# Autodesk Inventor assembly: chassis
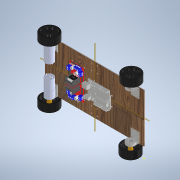
[picture p0: Inventor's stored thumbnail of the model, 180x180]
Saved by Autodesk Inventor 2022 (Build 260153000, 153)
## iProperties
Created: 2023-03-16
Part Number: chassis
Document SubType Name: Assembly
Designer: JOU
Author: JOU
## Documents named in this file (13)
- C:\Users\Johnny Jou\Documents\GitHub\Areo_Rider_Cabin\car\chassis.iam
- C:\Users\Johnny Jou\Documents\GitHub\Areo_Rider_Cabin\car\base.ipt
- C:\Users\Johnny Jou\Documents\GitHub\Areo_Rider_Cabin\car\motor_base.ipt
- C:\Users\Johnny Jou\Documents\GitHub\Areo_Rider_Cabin\motor\25GA370.ipt
- C:\Users\Johnny Jou\Documents\GitHub\Areo_Rider_Cabin\car\Coupling.ipt
- C:\Users\Johnny Jou\Documents\GitHub\Areo_Rider_Cabin\car\wheel.ipt
- C:\Users\Johnny Jou\Documents\GitHub\Areo_Rider_Cabin\car\chassis\機械便覽魔法師\軸承1.iam
- C:\Users\Johnny Jou\Documents\GitHub\Areo_Rider_Cabin\car\axle 4_20.ipt
- C:\Users\Johnny Jou\Documents\GitHub\Areo_Rider_Cabin\car\wheel_base.ipt
- C:\Users\Johnny Jou\Documents\GitHub\Areo_Rider_Cabin\car\wheel_base_cover.ipt
- C:\Users\Johnny Jou\Documents\GitHub\Areo_Rider_Cabin\car\arduino uno.ipt
- C:\Users\Johnny Jou\Documents\GitHub\Areo_Rider_Cabin\car\L298N.ipt
- C:\Users\Johnny Jou\Documents\GitHub\Areo_Rider_Cabin\car\bearing.iam
## Components (25 placed, 11 different names)
1. base:1 — 貼合:1, 貼合:2, 貼合:5, 貼合:6, 貼合:7, 貼合:8, 貼合:78, 貼合:79, 貼合:80, 貼合:81, 貼合:82, 貼合:83, 貼合:84, 貼合:85, 貼合:86, 貼合:87, 貼合:88, 貼合:89, 貼合:90, 貼合:91, 貼合:92
2. motor_base:1 — 貼合:1, 貼合:5, 貼合:6, 貼合:16, 貼合:17, 貼合:18
3. motor_base:2 — 貼合:2, 貼合:7, 貼合:8, 貼合:13, 貼合:14, 貼合:15
4. 25GA370:1 — 貼合:13, 貼合:14, 貼合:15, 貼合:33, 貼合:34
5. 25GA370:3 — 貼合:16, 貼合:17, 貼合:18, 貼合:22, 貼合:23
6. Coupling:1 — 貼合:19, 貼合:20, 貼合:21, 貼合:22, 貼合:23
7. wheel:1 — 貼合:19, 貼合:20, 貼合:21
8. Coupling:4 — 貼合:33, 貼合:34
9. wheel:4
10. Coupling:6 — 貼合:95
11. wheel:6
12. axle 4_20:3 — 貼合:93, 齊平:5
13. wheel_base:3 — 貼合:78, 貼合:82, 貼合:83
14. wheel_base_cover:3 — 貼合:94, 貼合:96
15. Coupling:7 — 貼合:98
16. wheel:7
17. 軸承:4 [sub-assembly]
18. axle 4_20:4 — 貼合:97, 齊平:6
19. wheel_base:4 — 貼合:79, 貼合:80, 貼合:81, 貼合:100, 貼合:102, 貼合:103
20. wheel_base_cover:4 — 貼合:99, 貼合:100, 貼合:101, 貼合:102, 貼合:103
21. arduino uno:1 — 貼合:84, 貼合:85, 貼合:86
22. L298N:1 — 貼合:87, 貼合:91, 貼合:92
23. L298N:2 — 貼合:88, 貼合:89, 貼合:90
24. 軸承:5 [sub-assembly] — 貼合:93, 齊平:5, 貼合:94, 貼合:95, 貼合:96
25. 軸承:6 [sub-assembly] — 貼合:97, 齊平:6, 貼合:98, 貼合:99, 貼合:101
## Relationships (65: Mate 62, Flush 3)
- 貼合:1 [Mate]: base:1 ↔ motor_base:1
- 貼合:2 [Mate]: base:1 ↔ motor_base:2
- 貼合:5 [Mate]: base:1 ↔ motor_base:1
- 貼合:6 [Mate]: base:1 ↔ motor_base:1
- 貼合:7 [Mate]: base:1 ↔ motor_base:2
- 貼合:8 [Mate]: base:1 ↔ motor_base:2
- 貼合:13 [Mate]: motor_base:2 ↔ 25GA370:1
- 貼合:14 [Mate]: motor_base:2 ↔ 25GA370:1
- 貼合:15 [Mate]: motor_base:2 ↔ 25GA370:1
- 貼合:16 [Mate]: motor_base:1 ↔ 25GA370:3
- 貼合:17 [Mate]: motor_base:1 ↔ 25GA370:3
- 貼合:18 [Mate]: motor_base:1 ↔ 25GA370:3
- 貼合:19 [Mate]: Coupling:1 ↔ wheel:1
- 貼合:20 [Mate]: Coupling:1 ↔ wheel:1
- 貼合:21 [Mate]: Coupling:1 ↔ wheel:1
- 貼合:22 [Mate]: 25GA370:3 ↔ Coupling:1
- 貼合:23 [Mate]: 25GA370:3 ↔ Coupling:1
- [Mate]: Coupling:4 ↔ wheel:4
- [Mate]: Coupling:4 ↔ wheel:4
- [Mate]: Coupling:4 ↔ wheel:4
- 貼合:33 [Mate]: 25GA370:1 ↔ Coupling:4
- 貼合:34 [Mate]: 25GA370:1 ↔ Coupling:4
- [Mate]: Coupling:6 ↔ wheel:6
- [Mate]: Coupling:6 ↔ wheel:6
- [Mate]: Coupling:6 ↔ wheel:6
- [Mate]: Coupling:6 ↔ axle 4_20:3
- [Mate]: Coupling:7 ↔ wheel:7
- [Mate]: Coupling:7 ↔ wheel:7
- [Mate]: Coupling:7 ↔ wheel:7
- [Mate]: Coupling:7 ↔ 軸承:4
- [Mate]: Coupling:7 ↔ axle 4_20:4
- [Flush]: 軸承:4 ↔ axle 4_20:4
- [Mate] (5 mm): Coupling:7 ↔ 軸承:4
- [Mate]: 軸承:4 ↔ wheel_base:4
- [Mate]: 軸承:4 ↔ wheel_base:4
- [Mate]: 軸承:4 ↔ wheel_base_cover:4
- [Mate]: 軸承:4 ↔ wheel_base_cover:4
- 貼合:78 [Mate]: base:1 ↔ wheel_base:3
- 貼合:79 [Mate]: base:1 ↔ wheel_base:4
- 貼合:80 [Mate]: base:1 ↔ wheel_base:4
- 貼合:81 [Mate]: base:1 ↔ wheel_base:4
- 貼合:82 [Mate]: base:1 ↔ wheel_base:3
- 貼合:83 [Mate]: base:1 ↔ wheel_base:3
- 貼合:84 [Mate] (5 mm): base:1 ↔ arduino uno:1
- 貼合:85 [Mate]: base:1 ↔ arduino uno:1
- 貼合:86 [Mate]: base:1 ↔ arduino uno:1
- 貼合:87 [Mate] (5 mm): base:1 ↔ L298N:1
- 貼合:88 [Mate] (5 mm): base:1 ↔ L298N:2
- 貼合:89 [Mate]: base:1 ↔ L298N:2
- 貼合:90 [Mate]: base:1 ↔ L298N:2
- 貼合:91 [Mate]: base:1 ↔ L298N:1
- 貼合:92 [Mate]: base:1 ↔ L298N:1
- 貼合:93 [Mate]: axle 4_20:3 ↔ 軸承:5
- 齊平:5 [Flush]: axle 4_20:3 ↔ 軸承:5
- 貼合:94 [Mate]: wheel_base_cover:3 ↔ 軸承:5
- 貼合:95 [Mate] (3 mm): Coupling:6 ↔ 軸承:5
- 貼合:96 [Mate]: wheel_base_cover:3 ↔ 軸承:5
- 貼合:97 [Mate]: axle 4_20:4 ↔ 軸承:6
- 齊平:6 [Flush]: axle 4_20:4 ↔ 軸承:6
- 貼合:98 [Mate] (3 mm): Coupling:7 ↔ 軸承:6
- 貼合:99 [Mate]: wheel_base_cover:4 ↔ 軸承:6
- 貼合:100 [Mate]: wheel_base:4 ↔ wheel_base_cover:4
- 貼合:101 [Mate]: wheel_base_cover:4 ↔ 軸承:6
- 貼合:102 [Mate]: wheel_base:4 ↔ wheel_base_cover:4
- 貼合:103 [Mate]: wheel_base:4 ↔ wheel_base_cover:4
## Named parameters: d32_d21 = 0 mm, d33_d22 = 0 mm, d34_d23 = 0 mm, d68_d26_d21 = 0 mm, d69_d27_d22 = 0 mm, d70_d28_d23 = 0 mm, d72_d38 = 0 mm, d74_d40 = 5 mm, d75_d41 = 0 mm, d76_d42 = 0 mm, d77_d43 = 0 mm, d78_d44 = 0 mm, d79_d26_d21 = 0 mm, d80_d27_d22 = 0 mm, d81_d28_d23 = 0 mm, d82_d37 = 0 mm, d83_d38 = 0 mm, d84_d39 = 0 mm
